# Autodesk Inventor assembly: lumped batteries
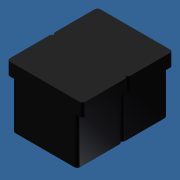
[picture p0: Inventor's stored thumbnail of the model, 180x180]
Saved by Autodesk Inventor 2012 (Build 160160000, 160)
## iProperties
Created: 2012-08-09
Part Number: lumped batteries
Document SubType Name: Assembly
Designer: Edward
Author: Edward
## Documents named in this file (2)
- C:\Users\Edward\Documents\masters\CAD\Invacare\lumped batteries.iam
- C:\Users\Edward\Documents\masters\CAD\Invacare\battery.ipt
## Components (2 placed, 1 different names)
1. battery:1 — Flush:1, Flush:2, Mate:1
2. battery:2 — Flush:1, Flush:2, Mate:1
## Relationships (3: Flush 2, Mate 1)
- Flush:1: battery:1 ↔ battery:2
- Flush:2: battery:1 ↔ battery:2
- Mate:1: battery:1 ↔ battery:2
